# Autodesk Inventor assembly: Assembly
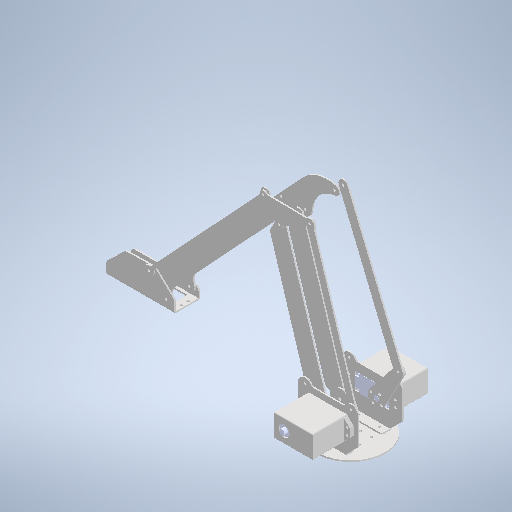
[picture p0: Inventor's stored thumbnail of the model, 512x512]
Saved by Autodesk Inventor 2025.2 (Build 292293000, 293)
## iProperties
Created: 2025-05-22
Part Number: Assembly
Document SubType Name: Assembly
Designer: Verchasv
Author: Verchasv
## Documents named in this file (16)
- C:\repo\Robotic-Arm\CAD\Assembly.iam
- C:\repo\Robotic-Arm\CAD\base plate.ipt
- C:\repo\Robotic-Arm\CAD\servo_holder_2.ipt
- C:\repo\Robotic-Arm\CAD\servo mount.ipt
- C:\repo\Robotic-Arm\CAD\Servo SC15.ipt
- C:\repo\Robotic-Arm\CAD\Arm 2\A2P1.ipt
- C:\repo\Robotic-Arm\CAD\Arm 2\A2P2.ipt
- C:\repo\Robotic-Arm\CAD\Arm 2\A2P3.ipt
- C:\repo\Robotic-Arm\CAD\Arm 1\A1P1.ipt
- C:\repo\Robotic-Arm\CAD\Arm 1\A1P2.ipt
- C:\repo\Robotic-Arm\CAD\Arm 1\A1P3.ipt
- C:\repo\Robotic-Arm\CAD\Arm 3\Arm 3 Part 1.ipt
- C:\repo\Robotic-Arm\CAD\Arm 3\Arm 3 Part 2.ipt
- C:\repo\Robotic-Arm\CAD\Arm 3\Arm 3 Part 3.ipt
- C:\repo\Robotic-Arm\CAD\Arm 2\A2P4.ipt
- C:\repo\Robotic-Arm\CAD\gripper servo mount.ipt
## Components (18 placed, 15 different names)
1. base plate:1 — Mate:1, Mate:2, Mate:3, Mate:8, Mate:9, Flush:2, Mate:20, Mate:21, Angle:10
2. servo_holder_2:1 — Mate:4, Mate:5, Mate:6, Mate:7, Angle:1, Flush:1
3. servo_holder_2:2 — Mate:10, Mate:11, Flush:3, Mate:12, Angle:2, Flush:4
4. servo mount:1 — Mate:1, Mate:2, Mate:3, Mate:4, Mate:5, Mate:6, Mate:13, Mate:14, Flush:5
5. servo mount:2 — Mate:8, Mate:9, Flush:2, Mate:10, Mate:11, Flush:3
6. Servo SC15:1 — Mate:12, Angle:2, Flush:4, Mate:17, Flush:10
7. Servo SC15:2 — Mate:7, Angle:1, Flush:1, Mate:23, Flush:7
8. A2P1:1 — Mate:13, Mate:14, Angle:11, Mate:40, Mate:42
9. A2P3:1 — Mate:31, Mate:32, Flush:9, Angle:12
10. A1P1:1 — Mate:17, Mate:18, Mate:36, Flush:10
11. A1P2:1 — Mate:18, Mate:19, Mate:36
12. A1P3:1 — Mate:19, Mate:25, Mate:27, Mate:30, Mate:37
13. Arm 3 Part 1:1 — Mate:25, Mate:27, Mate:28, Mate:29, Mate:37, Mate:39, Angle:12
14. Arm 3 Part 2:1 — Mate:22, Flush:6, Mate:38, Mate:39
15. Arm 3 Part 3:1 — Mate:20, Mate:21, Flush:5, Mate:22, Flush:6
16. A2P4:1 — Mate:23, Flush:7, Flush:9, Mate:38, Angle:11, Mate:41
17. gripper servo mount:1 — Mate:28, Mate:29, Mate:30, Mate:31, Mate:32, Angle:10
18. A2P2:1 — Mate:40, Mate:41, Mate:42
## Relationships (49: Mate 35, Flush 9, Angle 5)
- Mate:1: base plate:1 ↔ servo mount:1
- Mate:2: base plate:1 ↔ servo mount:1
- Mate:3: base plate:1 ↔ servo mount:1
- Mate:4: servo_holder_2:1 ↔ servo mount:1
- Mate:5: servo_holder_2:1 ↔ servo mount:1
- Mate:6: servo_holder_2:1 ↔ servo mount:1
- Mate:7: servo_holder_2:1 ↔ Servo SC15:2
- Angle:1 (0 deg): servo_holder_2:1 ↔ Servo SC15:2
- Flush:1: servo_holder_2:1 ↔ Servo SC15:2
- Mate:8: base plate:1 ↔ servo mount:2
- Mate:9: base plate:1 ↔ servo mount:2
- Flush:2 (-1.7 mm): base plate:1 ↔ servo mount:2
- Mate:10: servo_holder_2:2 ↔ servo mount:2
- Mate:11: servo_holder_2:2 ↔ servo mount:2
- Flush:3 (1.7 mm): servo_holder_2:2 ↔ servo mount:2
- Mate:12: servo_holder_2:2 ↔ Servo SC15:1
- Angle:2 (0 deg): servo_holder_2:2 ↔ Servo SC15:1
- Flush:4: servo_holder_2:2 ↔ Servo SC15:1
- Mate:13: servo mount:1 ↔ A2P1:1
- Mate:14: servo mount:1 ↔ A2P1:1
- Mate:17: Servo SC15:1 ↔ A1P1:1
- Mate:18: A1P1:1 ↔ A1P2:1
- Mate:19: A1P2:1 ↔ A1P3:1
- Mate:20: base plate:1 ↔ Arm 3 Part 3:1
- Mate:21: base plate:1 ↔ Arm 3 Part 3:1
- Flush:5: servo mount:1 ↔ Arm 3 Part 3:1
- Mate:22: Arm 3 Part 2:1 ↔ Arm 3 Part 3:1
- Flush:6 (-1.7 mm): Arm 3 Part 2:1 ↔ Arm 3 Part 3:1
- Mate:23: Servo SC15:2 ↔ A2P4:1
- Mate:25: A1P3:1 ↔ Arm 3 Part 1:1
- Mate:27: A1P3:1 ↔ Arm 3 Part 1:1
- Mate:28: Arm 3 Part 1:1 ↔ gripper servo mount:1
- Mate:29: Arm 3 Part 1:1 ↔ gripper servo mount:1
- Mate:30: A1P3:1 ↔ gripper servo mount:1
- Mate:31: A2P3:1 ↔ gripper servo mount:1
- Mate:32: A2P3:1 ↔ gripper servo mount:1
- Angle:10 (0 deg): base plate:1 ↔ gripper servo mount:1
- Flush:7: Servo SC15:2 ↔ A2P4:1
- Flush:9: A2P3:1 ↔ A2P4:1
- Mate:36: A1P1:1 ↔ A1P2:1
- Flush:10: Servo SC15:1 ↔ A1P1:1
- Mate:37: A1P3:1 ↔ Arm 3 Part 1:1
- Mate:38: Arm 3 Part 2:1 ↔ A2P4:1
- Mate:39: Arm 3 Part 1:1 ↔ Arm 3 Part 2:1
- Angle:11 (0 deg): A2P1:1 ↔ A2P4:1
- Mate:40: A2P1:1 ↔ A2P2:1
- Angle:12 (0 deg): A2P3:1 ↔ Arm 3 Part 1:1
- Mate:41: A2P4:1 ↔ A2P2:1
- Mate:42: A2P1:1 ↔ A2P2:1
